# Autodesk Inventor assembly: S6x2
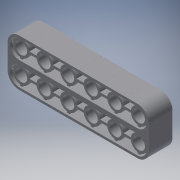
[picture p0: Inventor's stored thumbnail of the model, 180x180]
Saved by Autodesk Inventor 2019 (Build 230136000, 136)
## iProperties
Created: 2019-01-31
Part Number: S6x2
Document SubType Name: Assembly
Designer: Varga Daniel
Author: Varga Daniel
## Documents named in this file (4)
- C:\!_Dani\!_cloud\OneDrive\!_munka\Revolution\RevvyDemoKit\Structural parts\Straight Beams\S3+x2\S6x2.iam
- C:\!_Dani\!_cloud\OneDrive\!_munka\Revolution\RevvyDemoKit\Structural parts\Straight Beams\straight_beam_corner_part.ipt
- C:\!_Dani\!_cloud\OneDrive\!_munka\Revolution\RevvyDemoKit\Structural parts\Straight Beams\straight_beam_side_part.ipt
- C:\!_Dani\!_cloud\OneDrive\!_munka\Revolution\RevvyDemoKit\Structural parts\Straight Beams\S3+x2.iam
## Components (12 placed, 2 different names)
1. straight_beam_corner_part:1 — Flush:1, Flush:2, Mate:1, Flush:7, Mate:4, Flush:8, Flush:9, Mate:5, Flush:10
2. straight_beam_corner_part:2 — Flush:1, Flush:2, Mate:1
3. straight_beam_corner_part:3 — Flush:5, Flush:6, Mate:3, Flush:7, Mate:4, Flush:10
4. straight_beam_corner_part:4 — Flush:5, Flush:6, Mate:3
5. straight_beam_side_part:1 — Mate:2, Flush:3, Flush:4, Flush:8, Flush:9, Mate:5
6. straight_beam_side_part:2 — Mate:2, Flush:3, Flush:4
7. straight_beam_side_part:3
8. straight_beam_side_part:4
9. straight_beam_side_part:5
10. straight_beam_side_part:6
11. straight_beam_side_part:7
12. straight_beam_side_part:8
## Component patterns: (4 elements, first: straight_beam_side_part:1 + straight_beam_side_part:2)
## Relationships (15: Flush 10, Mate 5)
- Flush:1: straight_beam_corner_part:1 ↔ straight_beam_corner_part:2
- Flush:2: straight_beam_corner_part:1 ↔ straight_beam_corner_part:2
- Mate:1: straight_beam_corner_part:1 ↔ straight_beam_corner_part:2
- Mate:2: straight_beam_side_part:1 ↔ straight_beam_side_part:2
- Flush:3: straight_beam_side_part:1 ↔ straight_beam_side_part:2
- Flush:4: straight_beam_side_part:1 ↔ straight_beam_side_part:2
- Flush:5: straight_beam_corner_part:3 ↔ straight_beam_corner_part:4
- Flush:6: straight_beam_corner_part:3 ↔ straight_beam_corner_part:4
- Mate:3: straight_beam_corner_part:3 ↔ straight_beam_corner_part:4
- Flush:7: straight_beam_corner_part:1 ↔ straight_beam_corner_part:3
- Mate:4 (40 mm): straight_beam_corner_part:1 ↔ straight_beam_corner_part:3
- Flush:8: straight_beam_corner_part:1 ↔ straight_beam_side_part:1
- Flush:9: straight_beam_corner_part:1 ↔ straight_beam_side_part:1
- Mate:5: straight_beam_corner_part:1 ↔ straight_beam_side_part:1
- Flush:10: straight_beam_corner_part:1 ↔ straight_beam_corner_part:3
